# Autodesk Inventor assembly: Sample transfer
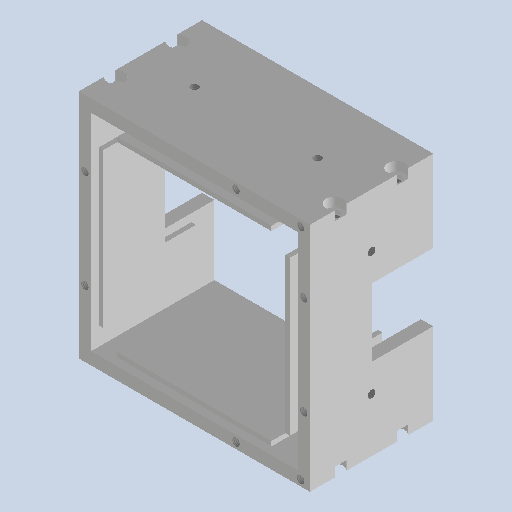
[picture p0: Inventor's stored thumbnail of the model, 512x512]
Saved by Autodesk Inventor 2026.1 (Build 301233000, 233)
## iProperties
Created: 2020-04-07
Part Number: Sample transfer
Document SubType Name: Assembly
Designer: Julian
Author: Julian
## Documents named in this file (6)
- C:\Users\user\Desktop\setup_inventor_2025\labjack\sample transfer neu\Sample transfer.iam
- C:\Users\user\Desktop\setup_inventor_2025\labjack\sample transfer neu\Left.ipt
- C:\Users\user\Desktop\setup_inventor_2025\labjack\sample transfer neu\Right.ipt
- C:\Users\user\Desktop\setup_inventor_2025\labjack\sample transfer neu\Front_Back.ipt
- C:\Users\user\Desktop\setup_inventor_2025\labjack\sample transfer neu\adapter plate.ipt
- C:\Users\user\Desktop\setup_inventor_2025\labjack\sample transfer neu\adapter plate_front back.ipt
## Components (8 placed, 5 different names)
1. Left:1 — Mate:7, Mate:8, Mate:9, Mate:12, Flush:2, Mate:13
2. Right:1 — Mate:1, Mate:2, Mate:3, Mate:4, Mate:5, Mate:6, Mate:10, Flush:1, Mate:11
3. Front_Back:1 — Mate:1, Mate:2, Mate:3, Mate:7, Mate:9, Mate:16, Flush:4, Mate:17
4. Front_Back:2 — Mate:4, Mate:5, Mate:6, Mate:8, Mate:14, Flush:3, Mate:15
5. adapter plate:1 — Mate:10, Flush:1, Mate:11
6. adapter plate:2 — Mate:12, Flush:2, Mate:13
7. adapter plate_front back:1 — Mate:14, Flush:3, Mate:15
8. adapter plate_front back:2 — Mate:16, Flush:4, Mate:17
## Relationships (21: Mate 17, Flush 4)
- Mate:1: Right:1 ↔ Front_Back:1
- Mate:2: Right:1 ↔ Front_Back:1
- Mate:3: Right:1 ↔ Front_Back:1
- Mate:4: Right:1 ↔ Front_Back:2
- Mate:5: Right:1 ↔ Front_Back:2
- Mate:6: Right:1 ↔ Front_Back:2
- Mate:7: Left:1 ↔ Front_Back:1
- Mate:8: Left:1 ↔ Front_Back:2
- Mate:9: Left:1 ↔ Front_Back:1
- Mate:10 (5 mm): Right:1 ↔ adapter plate:1
- Flush:1: Right:1 ↔ adapter plate:1
- Mate:11: Right:1 ↔ adapter plate:1
- Mate:12 (5 mm): Left:1 ↔ adapter plate:2
- Flush:2: Left:1 ↔ adapter plate:2
- Mate:13: Left:1 ↔ adapter plate:2
- Mate:14 (5 mm): Front_Back:2 ↔ adapter plate_front back:1
- Flush:3: Front_Back:2 ↔ adapter plate_front back:1
- Mate:15: Front_Back:2 ↔ adapter plate_front back:1
- Mate:16 (5 mm): Front_Back:1 ↔ adapter plate_front back:2
- Flush:4: Front_Back:1 ↔ adapter plate_front back:2
- Mate:17: Front_Back:1 ↔ adapter plate_front back:2
